# Autodesk Inventor assembly: GetriebeC
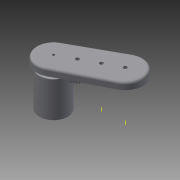
[picture p0: Inventor's stored thumbnail of the model, 180x180]
Saved by Autodesk Inventor 2014 (Build 180170000, 170)
## iProperties
Created: 2013-05-31
Part Number: GetriebeC
Document SubType Name: Assembly
Designer: hanse
Author: hanse
## Documents named in this file (7)
- C:\Users\Felix\Desktop\Beep\Hardware\GetriebeB\GetriebeC.iam
- C:\Users\Felix\Desktop\Beep\Hardware\GetriebeB\DoppelZahnrad.iam
- C:\Users\Felix\Desktop\Beep\Hardware\GetriebeB\Gertiebe\Konstruktions-Assistent\Stirnräder3.iam
- C:\Users\Felix\Desktop\Beep\Hardware\GetriebeB\BFront.ipt
- C:\Users\Felix\Desktop\Beep\Hardware\GetriebeB\EncoderWheel2.ipt
- C:\Users\Felix\Desktop\Beep\Hardware\EE-SX1131.ipt
- C:\Users\Felix\Desktop\Beep\Hardware\Model1\motor.ipt
## Components (8 placed, 6 different names)
1. Stirnräder:1 [sub-assembly] — Passend:8
2. DoppelZahnrad:1 [sub-assembly] — Passend:2, Passend:9
3. DoppelZahnrad:2 [sub-assembly] — Passend:2, Passend:3, Passend:10
4. DoppelZahnrad:3 [sub-assembly] — Passend:3, Passend:11
5. BFront:1
6. EncoderWheel2:1 — Passend:12, Passend:13
7. EE-SX1131:1 — Passend:12
8. motor:1 — Passend:14
## Relationships (9: Mate 9)
- Passend:2 [Mate] (15 mm): DoppelZahnrad:1 ↔ DoppelZahnrad:2
- Passend:3 [Mate] (15 mm): DoppelZahnrad:2 ↔ DoppelZahnrad:3
- Passend:8 [Mate]: Stirnräder:1
- Passend:9 [Mate]: DoppelZahnrad:1
- Passend:10 [Mate]: DoppelZahnrad:2
- Passend:11 [Mate]: DoppelZahnrad:3
- Passend:12 [Mate] (0.1 mm): EncoderWheel2:1 ↔ EE-SX1131:1
- Passend:13 [Mate]: EncoderWheel2:1
- Passend:14 [Mate]: motor:1
